# Autodesk Inventor assembly: Stewart-Plate-Inside
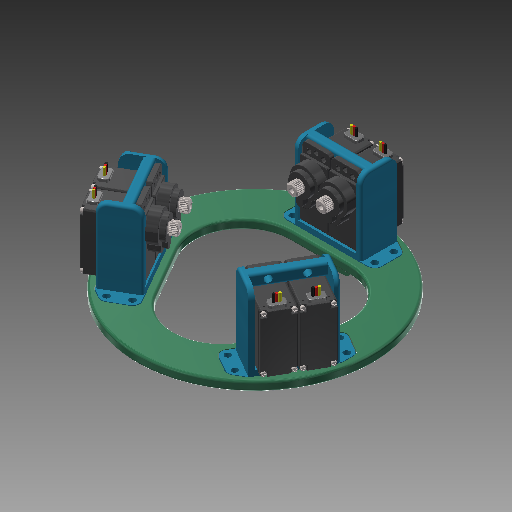
[picture p0: Inventor's stored thumbnail of the model, 512x512]
Saved by Autodesk Inventor 2018.2 (Build 222227000, 227)
## iProperties
Created: 2018-02-18
Part Number: Stewart-Plate-Inside
Material: Generisch
Document SubType Name: Assembly
Designer: JochenAlt
Author: JochenAlt
## Documents named in this file (4)
- D:\Projects\Donna\CAD\Stewart-Plate.iam
- D:\Projects\Donna\CAD\Stewart-Plate.ipt
- D:\Projects\Donna\CAD\Ball-Joint-male.ipt
- D:\Projects\Donna\CAD\Servo-Holder-Small.iam
## Components (10 placed, 3 different names)
1. Stewart-Plate:1 — Passend:1, Passend:2, Passend:3, Passend:4, Passend:5, Passend:6, Passend:7, Passend:8, Passend:9, Passend:10, Passend:11, Passend:12, Passend:13, Passend:14, Passend:15, Passend:16, Passend:17, Passend:18
2. ball joint:1 — Passend:2, Passend:9
3. ball joint:2 — Passend:4, Passend:12
4. ball joint:3 — Passend:5, Passend:8
5. ball joint:4 — Passend:6, Passend:7
6. ball joint:5 — Passend:3, Passend:11
7. ball joint:6 — Passend:1, Passend:10
8. Small-Servo-Holder:1 [sub-assembly] — Passend:13, Passend:14
9. Small-Servo-Holder:2 [sub-assembly] — Passend:15, Passend:16
10. Small-Servo-Holder:3 [sub-assembly] — Passend:17, Passend:18
## Relationships (18: Mate 18)
- Passend:1 [Mate]: Stewart-Plate:1 ↔ ball joint:6
- Passend:2 [Mate]: Stewart-Plate:1 ↔ ball joint:1
- Passend:3 [Mate]: Stewart-Plate:1 ↔ ball joint:5
- Passend:4 [Mate]: Stewart-Plate:1 ↔ ball joint:2
- Passend:5 [Mate]: Stewart-Plate:1 ↔ ball joint:3
- Passend:6 [Mate]: Stewart-Plate:1 ↔ ball joint:4
- Passend:7 [Mate]: Stewart-Plate:1 ↔ ball joint:4
- Passend:8 [Mate]: Stewart-Plate:1 ↔ ball joint:3
- Passend:9 [Mate]: Stewart-Plate:1 ↔ ball joint:1
- Passend:10 [Mate]: Stewart-Plate:1 ↔ ball joint:6
- Passend:11 [Mate]: Stewart-Plate:1 ↔ ball joint:5
- Passend:12 [Mate]: Stewart-Plate:1 ↔ ball joint:2
- Passend:13 [Mate]: Stewart-Plate:1 ↔ Small-Servo-Holder:1
- Passend:14 [Mate]: Stewart-Plate:1 ↔ Small-Servo-Holder:1
- Passend:15 [Mate]: Stewart-Plate:1 ↔ Small-Servo-Holder:2
- Passend:16 [Mate]: Stewart-Plate:1 ↔ Small-Servo-Holder:2
- Passend:17 [Mate]: Stewart-Plate:1 ↔ Small-Servo-Holder:3
- Passend:18 [Mate]: Stewart-Plate:1 ↔ Small-Servo-Holder:3
